# Autodesk Inventor assembly: SansCapacFata
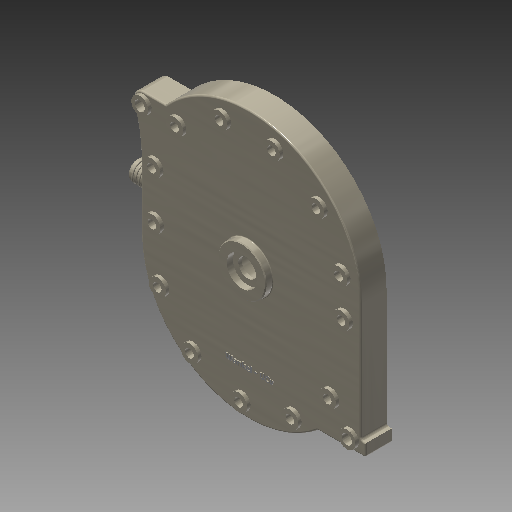
[picture p0: Inventor's stored thumbnail of the model, 512x512]
Saved by Autodesk Inventor 2019.4 (Build 234330000, 330)
## iProperties
Created: 2020-05-01
Part Number: SansCapacFata
Document SubType Name: Assembly
Designer: Gabriel
Author: Gabriel
## Documents named in this file (4)
- C:\Users\Gabriel\Desktop\Teme Gac\MotorWankel\SansCapacFata.iam
- C:\Users\Gabriel\Desktop\Teme Gac\MotorWankel\CapacFata.ipt
- C:\Users\Gabriel\Desktop\Teme Gac\MotorWankel\Spur Gear11.ipt
- C:\Users\Gabriel\Desktop\Teme Gac\MotorWankel\SubansM4x10.iam
## Components (3 placed, 3 different names)
1. CapacFata:1 — Mate:1, Mate:2, Angle:1
2. Spur Gear1:1 — Mate:1, Mate:2, Angle:1
3. SubansM4x10:1 [sub-assembly]
## Relationships (4: Mate 2, Angle 1, Insert 1)
- Mate:1: CapacFata:1 ↔ Spur Gear1:1
- Mate:2: CapacFata:1 ↔ Spur Gear1:1
- Angle:1 (99 deg): CapacFata:1 ↔ Spur Gear1:1
- [Insert]: Spur Gear1:1 ↔ SubansM4x10:1
